# Autodesk Inventor assembly: Assy_cover_front
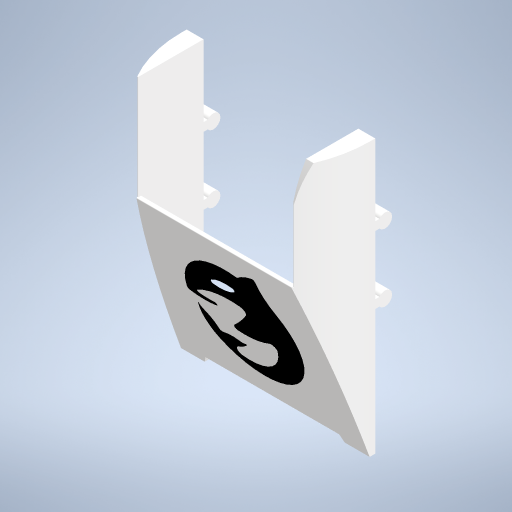
[picture p0: Inventor's stored thumbnail of the model, 512x512]
Saved by Autodesk Inventor 2024.1 (Build 281209000, 209)
## iProperties
Created: 2025-03-07
Part Number: Assy_cover_front
Document SubType Name: Assembly
Designer: hibik
Author: hibik
## Documents named in this file (3)
- C:\Users\hibik\Documents\Robomech\RESCUE\ORCA\hard\cover\Assy_cover_front.iam
- C:\Users\hibik\Documents\Robomech\RESCUE\ORCA\hard\cover\cover_front.ipt
- C:\Users\hibik\Documents\Robomech\RESCUE\ORCA\hard\cover\ROGO_front_cover.ipt
## Components (2 placed, 2 different names)
1. cover_front:1 — フラッシュ:3
2. ROGO_front_cover:1 — フラッシュ:2, フラッシュ:3
## Relationships (2: Flush 2)
- フラッシュ:2 [Flush]: ROGO_front_cover:1
- フラッシュ:3 [Flush] (30 mm): cover_front:1 ↔ ROGO_front_cover:1
